# Autodesk Inventor assembly: Assembly1
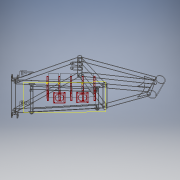
[picture p0: Inventor's stored thumbnail of the model, 180x180]
Saved by Autodesk Inventor 2019.3 (Build 233278000, 278)
## iProperties
Created: 2019-03-03
Part Number: Assembly1
Document SubType Name: Assembly
Designer: eroldan
Author: eroldan
## Documents named in this file (6)
- C:\Users\eroldan\Desktop\3dprojects\OpenEmoto\MainFrame\Battery2\Assembly1.iam
- C:\Users\eroldan\Desktop\3dprojects\OpenEmoto\MainFrame\MainFrame.ipt
- C:\Users\eroldan\Desktop\3dprojects\OpenEmoto\MainFrame\Battery\LowerCage.ipt
- C:\Users\eroldan\Desktop\3dprojects\OpenEmoto\MainFrame\Battery2\Zippy-5S-5Ah.ipt
- C:\Users\eroldan\Desktop\3dprojects\OpenEmoto\MainFrame\Battery\SpacerBig.ipt
- C:\Users\eroldan\Desktop\3dprojects\OpenEmoto\MainFrame\Battery\SpacerSmall.ipt
## Components (13 placed, 5 different names)
1. MainFrame:1
2. LowerCage:1 — Flush:1, Mate:13, Mate:14, Mate:15, Mate:16, Mate:17, Mate:18, Mate:19, Mate:20, Mate:21, Mate:22, Mate:23
3. Zippy-5S-5Ah:1 — Flush:2, Mate:1, Mate:9, Mate:20
4. SpacerBig:1 — Mate:1, Mate:2, Mate:14
5. Zippy-5S-5Ah:2 — Mate:2, Flush:3, Mate:3, Mate:12, Mate:21
6. SpacerBig:2 — Mate:3, Mate:4, Mate:15
7. Zippy-5S-5Ah:3 — Mate:4, Flush:4, Mate:6, Mate:11, Mate:22
8. SpacerBig:3 — Mate:6, Mate:7, Mate:16
9. Zippy-5S-5Ah:4 — Mate:7, Flush:5, Mate:8, Mate:23
10. SpacerBig:4 — Mate:8, Mate:17
11. SpacerBig:5 — Mate:9, Mate:13
12. SpacerSmall:2 — Mate:11, Mate:18
13. SpacerSmall:3 — Mate:12, Mate:19
## Relationships (26: Mate 21, Flush 5)
- Flush:1 (-15 mm): LowerCage:1
- Flush:2: Zippy-5S-5Ah:1
- Mate:1: Zippy-5S-5Ah:1 ↔ SpacerBig:1
- Mate:2: SpacerBig:1 ↔ Zippy-5S-5Ah:2
- Flush:3: Zippy-5S-5Ah:2
- Mate:3: Zippy-5S-5Ah:2 ↔ SpacerBig:2
- Mate:4: SpacerBig:2 ↔ Zippy-5S-5Ah:3
- Flush:4: Zippy-5S-5Ah:3
- Mate:6: Zippy-5S-5Ah:3 ↔ SpacerBig:3
- Mate:7: SpacerBig:3 ↔ Zippy-5S-5Ah:4
- Flush:5: Zippy-5S-5Ah:4
- Mate:8: Zippy-5S-5Ah:4 ↔ SpacerBig:4
- Mate:9: Zippy-5S-5Ah:1 ↔ SpacerBig:5
- Mate:11: Zippy-5S-5Ah:3 ↔ SpacerSmall:2
- Mate:12: Zippy-5S-5Ah:2 ↔ SpacerSmall:3
- Mate:13: LowerCage:1 ↔ SpacerBig:5
- Mate:14: LowerCage:1 ↔ SpacerBig:1
- Mate:15: LowerCage:1 ↔ SpacerBig:2
- Mate:16: LowerCage:1 ↔ SpacerBig:3
- Mate:17: LowerCage:1 ↔ SpacerBig:4
- Mate:18: LowerCage:1 ↔ SpacerSmall:2
- Mate:19: LowerCage:1 ↔ SpacerSmall:3
- Mate:20: LowerCage:1 ↔ Zippy-5S-5Ah:1
- Mate:21: LowerCage:1 ↔ Zippy-5S-5Ah:2
- Mate:22: LowerCage:1 ↔ Zippy-5S-5Ah:3
- Mate:23: LowerCage:1 ↔ Zippy-5S-5Ah:4
